# Autodesk Inventor assembly: High Strength 60-tooth Gear-Square Insert
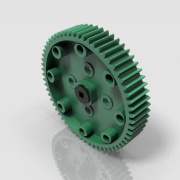
[picture p0: Inventor's stored thumbnail of the model, 180x180]
Saved by Autodesk Inventor 2013 (Build 170138000, 138)
## iProperties
Category: Motion
Company: Super Sonic Sparks, Team 24
Document SubType Name: Assembly
Designer: Jordan Kiesel
Vendor: VEX Robotics, Inc.
Description: Metal Square Hole Inserts prevent axles from "stripping".
Catalog Web Link: http://www.vexrobotics.com/products/accessories/motion/276-2250.html
Author: Jordan Kiesel
Title: High Strength 60-tooth Gear-Square Insert
Comments: Build mechanisms capable of withstanding higher stresses than ever before. Lift heavier loads, and survive bigger impacts with high strength gears. ▷ High strength gears mate with all VEX spur gears. ▷ Double-thick face width provides added tooth strength. ▷ Metal Square Hole Inserts prevent axles from "stripping". ▷ Build gearboxes that resist high shock-loads. ▷ Bolt Gears together for added strength.
## Documents named in this file (3)
- C:\Users\WEBCAST2\Documents\New VEX CAD Parts\Spur Gears\High Strength 60-tooth Gear-Square Insert.iam
- C:\Users\WEBCAST2\Documents\New VEX CAD Parts\Spur Gears\Assembly Parts\High Strength Gears\High Strength 60-Tooth Gear.ipt
- C:\Users\WEBCAST2\Documents\New VEX CAD Parts\Spur Gears\Assembly Parts\High Strength Gears\High Strength Square Gear Insert.ipt
## Components (3 placed, 2 different names)
1. High Strength 60-Tooth Gear:1 — Mate:1, Mate:2, Mate:3, Mate:4, Mate:5, Mate:6
2. High Strength Square Gear Insert:1 — Mate:1, Mate:2, Mate:3
3. High Strength Square Gear Insert:2 — Mate:4, Mate:5, Mate:6
## Relationships (6: Mate 6)
- Mate:1: High Strength 60-Tooth Gear:1 ↔ High Strength Square Gear Insert:1
- Mate:2 (0.0254 mm): High Strength 60-Tooth Gear:1 ↔ High Strength Square Gear Insert:1
- Mate:3 (0.0254 mm): High Strength 60-Tooth Gear:1 ↔ High Strength Square Gear Insert:1
- Mate:4: High Strength 60-Tooth Gear:1 ↔ High Strength Square Gear Insert:2
- Mate:5 (0.0254 mm): High Strength 60-Tooth Gear:1 ↔ High Strength Square Gear Insert:2
- Mate:6 (0.0254 mm): High Strength 60-Tooth Gear:1 ↔ High Strength Square Gear Insert:2
